# Autodesk Inventor assembly: LCD+Case
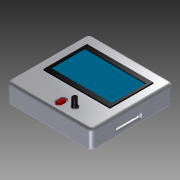
[picture p0: Inventor's stored thumbnail of the model, 180x180]
Saved by Autodesk Inventor 2016 (Build 200138000, 138)
## iProperties
Created: 2015-04-16
Part Number: LCD+Case
Document SubType Name: Assembly
Designer: Jack
Author: Jack
## Documents named in this file (5)
- C:\Users\Jack\ownCloud\Projects\CrossBot\InventorModel\Enclosure\LCDCase\LCD+Case.iam
- C:\Users\Jack\ownCloud\Projects\CrossBot\InventorModel\Electronics\LCD\GLCDKnockoff.ipt
- C:\Users\Jack\ownCloud\Projects\CrossBot\InventorModel\Enclosure\LCDCase\LCDDerivativeBottom1.ipt
- C:\Users\Jack\ownCloud\Projects\CrossBot\InventorModel\Enclosure\LCDCase\LCDDerivativeTop1.ipt
- C:\Users\Jack\ownCloud\Projects\CrossBot\InventorModel\Enclosure\LCDCase\LCDButton.ipt
## Components (4 placed, 4 different names)
1. GLCDKnockoff:1 — Mate:3, Mate:4, Mate:5, Mate:6, Mate:11, Mate:12, Mate:13, Mate:17, Mate:23
2. LCDDerivativeBottom1:1 — Mate:11, Mate:12, Mate:13, Mate:23
3. LCDDerivativeTop1:1 — Mate:3, Mate:4, Mate:5, Mate:6, Mate:14, Mate:17, Mate:18, Angle:1
4. LCDButton:1 — Mate:14, Mate:18, Angle:1
## Relationships (12: Mate 11, Angle 1)
- Mate:3: GLCDKnockoff:1 ↔ LCDDerivativeTop1:1
- Mate:4: GLCDKnockoff:1 ↔ LCDDerivativeTop1:1
- Mate:5: GLCDKnockoff:1 ↔ LCDDerivativeTop1:1
- Mate:6: GLCDKnockoff:1 ↔ LCDDerivativeTop1:1
- Mate:11: GLCDKnockoff:1 ↔ LCDDerivativeBottom1:1
- Mate:12: GLCDKnockoff:1 ↔ LCDDerivativeBottom1:1
- Mate:13: GLCDKnockoff:1 ↔ LCDDerivativeBottom1:1
- Mate:14: LCDDerivativeTop1:1 ↔ LCDButton:1
- Mate:17: GLCDKnockoff:1 ↔ LCDDerivativeTop1:1
- Mate:18: LCDDerivativeTop1:1 ↔ LCDButton:1
- Mate:23: GLCDKnockoff:1 ↔ LCDDerivativeBottom1:1
- Angle:1 (180 deg): LCDDerivativeTop1:1 ↔ LCDButton:1
